# Autodesk Inventor assembly: Assembly_Test
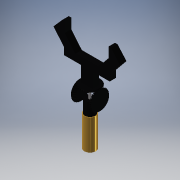
[picture p0: Inventor's stored thumbnail of the model, 180x180]
Saved by Autodesk Inventor 2016 (Build 200138000, 138)
## iProperties
Created: 2015-05-21
Part Number: Assembly_Test
Document SubType Name: Assembly
Designer: CHUNGBK
Mass: 1018 g
Surface Area: 473.269 cm^2
Volume: 188.163 cm^3
Author: CHUNGBK
## Documents named in this file (5)
- C:\Users\jonathan\Documents\GitHub\Integrated-Tool-Suite\Five Axis Serial Robotic Arm\Inventor\Gripper Assembly.iam
- C:\Users\jonathan\Documents\GitHub\Integrated-Tool-Suite\Five Axis Serial Robotic Arm\Inventor\Gripper Motor.ipt
- C:\Users\jonathan\Documents\GitHub\Integrated-Tool-Suite\Five Axis Serial Robotic Arm\Inventor\Bevel Gear.ipt
- C:\Users\jonathan\Documents\GitHub\Integrated-Tool-Suite\Five Axis Serial Robotic Arm\Inventor\Gripper Gear.ipt
- C:\Users\jonathan\Documents\GitHub\Integrated-Tool-Suite\Five Axis Serial Robotic Arm\Inventor\Motor Shaft.ipt
## Components (5 placed, 3 different names)
1. Gripper Motor:1 — Mate:5, Mate:6
2. Bevel Gear1:1 — Mate:14, Angle:1, Angle:4
3. Bevel Gear1:2 — Mate:13, Mate:14, Angle:1, Angle:2, Angle:3
4. Bevel Gear1:3 — Mate:7, Mate:8, Flush:1, Flush:2, Mate:12, Mate:13, Angle:2, Angle:3, Angle:4
5. Motor Shaft:1 — Mate:5, Mate:6, Mate:7, Mate:8
## Relationships (13: Mate 7, Angle 4, Flush 2)
- Mate:5: Gripper Motor:1 ↔ Motor Shaft:1
- Mate:6: Gripper Motor:1 ↔ Motor Shaft:1
- Mate:7: Bevel Gear1:3 ↔ Motor Shaft:1
- Mate:8: Bevel Gear1:3 ↔ Motor Shaft:1
- Flush:1: Bevel Gear1:3
- Flush:2: Bevel Gear1:3
- Mate:12: Bevel Gear1:3
- Mate:13: Bevel Gear1:2 ↔ Bevel Gear1:3
- Mate:14: Bevel Gear1:1 ↔ Bevel Gear1:2
- Angle:1 (180 deg): Bevel Gear1:1 ↔ Bevel Gear1:2
- Angle:2 (90 deg): Bevel Gear1:2 ↔ Bevel Gear1:3
- Angle:3 (0 deg): Bevel Gear1:2 ↔ Bevel Gear1:3
- Angle:4 (0 deg): Bevel Gear1:1 ↔ Bevel Gear1:3
